# Autodesk Inventor assembly: GFRP_T2_17
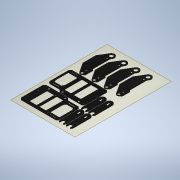
[picture p0: Inventor's stored thumbnail of the model, 180x180]
Saved by Autodesk Inventor 2020 (Build 240168000, 168)
## iProperties
Created: 2021-08-27
Part Number: GFRP_T2_17
Document SubType Name: Assembly
Designer: Masato
Author: Masato
## Documents named in this file (5)
- C:\Inventor\SUSTAINA-OP\Cam\GFRP_T2_17.iam
- C:\Inventor\SUSTAINA-OP\Cam\DisposableBoard.ipt
- C:\Inventor\SUSTAINA-OP\UpperBody\Trunk\Trunk_upper_side_frame.ipt
- C:\Inventor\SUSTAINA-OP\LowerBody\Link\FrontLink_frame.ipt
- C:\Inventor\SUSTAINA-OP\UpperBody\Arm\ForeArm_inside_frame.ipt
## Components (11 placed, 4 different names)
1. DisposableBoard:1 — メイト:2, メイト:1, フラッシュ:1, フラッシュ:2, メイト:4, メイト:5, フラッシュ:3, フラッシュ:4, メイト:15, フラッシュ:6, メイト:16, 正接:4
2. Trunk_upper_side_frame:1 — メイト:4, フラッシュ:3, フラッシュ:4, メイト:6, フラッシュ:5, メイト:17
3. Trunk_upper_side_frame:2 — メイト:5, メイト:6, フラッシュ:5, 正接:3
4. FrontLink_frame:1 — メイト:15, 正接:3, フラッシュ:6
5. FrontLink_frame:2
6. FrontLink_frame:3
7. FrontLink_frame:4
8. ForeArm_inside_frame:1 — メイト:16, 正接:4, メイト:17
9. ForeArm_inside_frame:2
10. ForeArm_inside_frame:3
11. ForeArm_inside_frame:4
## Component patterns: (4 elements, first: FrontLink_frame:1), (4 elements, first: ForeArm_inside_frame:1)
## Relationships (16: Mate 8, Flush 6, Tangent 2)
- メイト:2 [Mate]: DisposableBoard:1
- メイト:1 [Mate]: DisposableBoard:1
- フラッシュ:1 [Flush]: DisposableBoard:1
- フラッシュ:2 [Flush]: DisposableBoard:1
- メイト:4 [Mate]: DisposableBoard:1 ↔ Trunk_upper_side_frame:1
- メイト:5 [Mate]: DisposableBoard:1 ↔ Trunk_upper_side_frame:2
- フラッシュ:3 [Flush] (-2.5 mm): DisposableBoard:1 ↔ Trunk_upper_side_frame:1
- フラッシュ:4 [Flush] (2.5 mm): DisposableBoard:1 ↔ Trunk_upper_side_frame:1
- メイト:6 [Mate] (2.5 mm): Trunk_upper_side_frame:1 ↔ Trunk_upper_side_frame:2
- フラッシュ:5 [Flush]: Trunk_upper_side_frame:1 ↔ Trunk_upper_side_frame:2
- メイト:15 [Mate]: DisposableBoard:1 ↔ FrontLink_frame:1
- 正接:3 [Tangent] (2.5 mm): Trunk_upper_side_frame:2 ↔ FrontLink_frame:1
- フラッシュ:6 [Flush] (5 mm): DisposableBoard:1 ↔ FrontLink_frame:1
- メイト:16 [Mate]: DisposableBoard:1 ↔ ForeArm_inside_frame:1
- 正接:4 [Tangent] (2 mm): DisposableBoard:1 ↔ ForeArm_inside_frame:1
- メイト:17 [Mate] (2.5 mm): Trunk_upper_side_frame:1 ↔ ForeArm_inside_frame:1
